# Autodesk Inventor assembly: DD_KVD_002_B
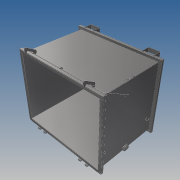
[picture p0: Inventor's stored thumbnail of the model, 180x180]
Saved by Autodesk Inventor 2017.3 (Build 213256000, 256)
## iProperties
Created: 2023-12-07
Part Number: DD_KVD_002_B
Document SubType Name: Weldment
Designer: Darena
Weld Material: Nerezová ocel, kartáčovaná
Author: Darena
## Documents named in this file (18)
- D:\2_Darena\1_Soukrome\02_Inventor soukromé\Dílna RAKO3\Záhora\Pivovar KONTEJNER\S výklopným dnem\DD_KVD_001\DD_KVD_002_B.iam
- D:\2_Darena\1_Soukrome\02_Inventor soukromé\Dílna RAKO3\Záhora\Pivovar KONTEJNER\S výklopným dnem\DD_KVD_001\DD_KVD_002_01.ipt
- D:\2_Darena\1_Soukrome\02_Inventor soukromé\Dílna RAKO3\Záhora\Pivovar KONTEJNER\S výklopným dnem\DD_KVD_001\DD_KVD_002_02.ipt
- D:\2_Darena\1_Soukrome\02_Inventor soukromé\Dílna RAKO3\Záhora\Pivovar KONTEJNER\S výklopným dnem\DD_KVD_001\DD_KVD_002_05.ipt
- D:\2_Darena\1_Soukrome\02_Inventor soukromé\Dílna RAKO3\Záhora\Pivovar KONTEJNER\S výklopným dnem\DD_KVD_001\DD_KVD_002_03.ipt
- D:\2_Darena\1_Soukrome\02_Inventor soukromé\Dílna RAKO3\Záhora\Pivovar KONTEJNER\S výklopným dnem\DD_KVD_001\DD_KVD_002_04.ipt
- D:\2_Darena\1_Soukrome\02_Inventor soukromé\Dílna RAKO3\Záhora\Pivovar KONTEJNER\S výklopným dnem\DD_KVD_001\DD_KVD_003_10_A.ipt
- D:\2_Darena\1_Soukrome\02_Inventor soukromé\Dílna RAKO3\Záhora\Pivovar KONTEJNER\S výklopným dnem\DD_KVD_001\DD_KVD_002_06.ipt
- D:\2_Darena\1_Soukrome\02_Inventor soukromé\Dílna RAKO3\Záhora\Pivovar KONTEJNER\S výklopným dnem\DD_KVD_001\DD_KVD_002_07.ipt
- D:\2_Darena\1_Soukrome\02_Inventor soukromé\Dílna RAKO3\Záhora\Pivovar KONTEJNER\S výklopným dnem\DD_KVD_001\DD_KVD_002_08.ipt
- D:\2_Darena\1_Soukrome\02_Inventor soukromé\Dílna RAKO3\Záhora\Pivovar KONTEJNER\S výklopným dnem\DD_KVD_001\DD_KVD_002_09.ipt
- D:\2_Darena\1_Soukrome\02_Inventor soukromé\Dílna RAKO3\Záhora\Pivovar KONTEJNER\S výklopným dnem\DD_KVD_001\DD_KVD_002_10.ipt
- D:\2_Darena\1_Soukrome\02_Inventor soukromé\Dílna RAKO3\Záhora\Pivovar KONTEJNER\S výklopným dnem\DD_KVD_001\DD_KVD_002_11.ipt
- D:\2_Darena\1_Soukrome\02_Inventor soukromé\Dílna RAKO3\Záhora\Pivovar KONTEJNER\S výklopným dnem\DD_KVD_001\ZA_VK_010.iam
- D:\2_Darena\1_Soukrome\02_Inventor soukromé\Dílna RAKO3\Záhora\Pivovar KONTEJNER\S výklopným dnem\DD_KVD_001\DD_KVD_002_13.ipt
- D:\2_Darena\1_Soukrome\02_Inventor soukromé\Dílna RAKO3\Záhora\Pivovar KONTEJNER\S výklopným dnem\DD_KVD_001\DD_KVD_002_12.ipt
- D:\2_Darena\1_Soukrome\02_Inventor soukromé\Dílna RAKO3\Záhora\Pivovar KONTEJNER\S výklopným dnem\DD_KVD_001\DD_KVD_002_14.ipt
- D:\2_Darena\1_Soukrome\02_Inventor soukromé\Dílna RAKO3\Záhora\Pivovar KONTEJNER\S výklopným dnem\DD_KVD_001\DD_KVD_004.iam
## Components (38 placed, 17 different names)
1. DD_KVD_002_01:1 — Stejný směr:7, Proti sobě:65, Proti sobě:69, Proti sobě:71, Proti sobě:72, Stejný směr:11, Stejný směr:12, Proti sobě:84, Proti sobě:86, Stejný směr:21, Proti sobě:101, Proti sobě:103, Proti sobě:105, Stejný směr:29, Proti sobě:128, Úhel:7
2. DD_KVD_002_01:2 — Proti sobě:63, Proti sobě:66, Proti sobě:67, Proti sobě:74, Stejný směr:13, Proti sobě:121, Proti sobě:124, Stejný směr:32, Stejný směr:39
3. DD_KVD_002_02:2 — Stejný směr:6, Proti sobě:65, Proti sobě:66, Stejný směr:12, Stejný směr:13, Proti sobě:90, Proti sobě:118, Proti sobě:122, Stejný směr:31, Proti sobě:130, Proti sobě:132, Proti sobě:133
4. DD_KVD_002_02:3 — Proti sobě:64, Proti sobě:67, Proti sobě:70, Stejný směr:11, Úhel:3, Úhel:4, Proti sobě:127, Proti sobě:131
5. DD_KVD_002_03:1 — Stejný směr:3, Proti sobě:57, Proti sobě:58, Stejný směr:4, Proti sobě:59
6. DD_KVD_002_03:2 — Stejný směr:5, Proti sobě:61, Proti sobě:62, Proti sobě:70
7. DD_KVD_002_03:3 — Stejný směr:17, Proti sobě:90, Proti sobě:97, Stejný směr:23, Proti sobě:129, Proti sobě:134
8. DD_KVD_002_03:4 — Proti sobě:85, Stejný směr:16, Proti sobě:99, Stejný směr:24, Stejný směr:33, Stejný směr:36
9. DD_KVD_002_04:1 — Stejný směr:4, Proti sobě:59, Stejný směr:5, Proti sobě:75, Proti sobě:123, Proti sobě:126
10. DD_KVD_002_04:2 — Stejný směr:3, Proti sobě:57, Proti sobě:58, Proti sobě:61, Proti sobě:62, Proti sobě:69, Proti sobě:71, Proti sobě:73
11. DD_KVD_002_04:3 — Proti sobě:91, Proti sobě:92, Proti sobě:93, Proti sobě:94, Proti sobě:95, Stejný směr:37
12. DD_KVD_002_04:4 — Proti sobě:84, Proti sobě:85, Stejný směr:16, Stejný směr:17, Proti sobě:86, Proti sobě:100, Proti sobě:102, Proti sobě:104, HÁK ZAJIŠTĚNÝ, Proti sobě:119
13. DD_KVD_003_10_A:1 — Proti sobě:91, Stejný směr:20, Proti sobě:95, Proti sobě:96
14. DD_KVD_003_10_A:2 — Proti sobě:92, Stejný směr:19, Stejný směr:20, Proti sobě:96, Proti sobě:97
15. DD_KVD_003_10_A:3 — Proti sobě:93, Stejný směr:18, Proti sobě:98
16. DD_KVD_003_10_A:4 — Proti sobě:94, Stejný směr:18, Stejný směr:19, Proti sobě:98, Proti sobě:99
17. DD_KVD_002_06:1 — Proti sobě:100, Proti sobě:101, Stejný směr:23, Proti sobě:106, Proti sobě:107
18. DD_KVD_002_06:2 — Stejný směr:22, Proti sobě:102, Proti sobě:103, Proti sobě:110
19. DD_KVD_002_06:3 — Proti sobě:104, Proti sobě:105, Stejný směr:24, Proti sobě:108, Proti sobě:109
20. DD_KVD_002_07:1 — Proti sobě:106, Proti sobě:107, Stejný směr:25, Úhel:1, HÁK ZAJIŠTĚNÝ, Úhel:5
21. DD_KVD_002_07:2 — Proti sobě:108, Proti sobě:109, Stejný směr:25, Úhel:2
22. DD_KVD_002_08:1 — Proti sobě:110, Stejný směr:26, Úhel:1, Proti sobě:112, Stejný směr:27, Proti sobě:113, Stejný směr:28
23. DD_KVD_002_09:1 — Proti sobě:112, Stejný směr:27, Úhel:5, Úhel:6
24. DD_KVD_002_10:1 — Proti sobě:113, Stejný směr:28, Úhel:2
25. ZA_VK_010:1 [sub-assembly] — Úhel:3, Úhel:4, Tečnost:4, Stejný směr:34
26. DD_KVD_002_13:1 — Proti sobě:118, Proti sobě:119, Stejný směr:29, Proti sobě:120, Tečnost:3
27. DD_KVD_002_12:1 — Proti sobě:120, Tečnost:3, Úhel:6, Proti sobě:132, Úhel:7
28. DD_KVD_002_14:1 — Proti sobě:124, Proti sobě:125, Proti sobě:126, Stejný směr:30
29. DD_KVD_002_14:2 — Stejný směr:30, Stejný směr:31, Stejný směr:32
30. DD_KVD_002_14:3 — Proti sobě:121, Proti sobě:122, Proti sobě:123, Proti sobě:125
31. DD_KVD_002_11:1 — Proti sobě:127, Proti sobě:128, Stejný směr:33, Tečnost:4, Stejný směr:34
32. DD_KVD_002_14:4 — Stejný směr:36, Proti sobě:131, Stejný směr:37, Stejný směr:38
33. DD_KVD_002_14:5 — Proti sobě:129, Proti sobě:130, Stejný směr:38
34. DD_KVD_004:1 [sub-assembly] — Proti sobě:133, Stejný směr:39, Proti sobě:134
35. DD_KVD_002_05:5 — Proti sobě:72, Proti sobě:73, Stejný směr:9, Stejný směr:10
36. DD_KVD_002_05:6 — Proti sobě:74, Proti sobě:75, Stejný směr:9
37. DD_KVD_002_05:7
38. DD_KVD_002_05:8
## Component patterns: (2 elements, first: DD_KVD_002_05:5 + DD_KVD_002_05:6)
## Relationships (108: Mate 64, Flush 35, Angle 7, Tangent 2)
- Proti sobě:63 [Mate]: DD_KVD_002_01:2
- Stejný směr:3 [Flush]: DD_KVD_002_03:1 ↔ DD_KVD_002_04:2
- Proti sobě:57 [Mate]: DD_KVD_002_03:1 ↔ DD_KVD_002_04:2
- Proti sobě:58 [Mate]: DD_KVD_002_03:1 ↔ DD_KVD_002_04:2
- Stejný směr:4 [Flush]: DD_KVD_002_03:1 ↔ DD_KVD_002_04:1
- Proti sobě:59 [Mate]: DD_KVD_002_03:1 ↔ DD_KVD_002_04:1
- Stejný směr:5 [Flush]: DD_KVD_002_03:2 ↔ DD_KVD_002_04:1
- Proti sobě:61 [Mate]: DD_KVD_002_03:2 ↔ DD_KVD_002_04:2
- Proti sobě:62 [Mate]: DD_KVD_002_03:2 ↔ DD_KVD_002_04:2
- Proti sobě:64 [Mate]: DD_KVD_002_02:3
- Stejný směr:6 [Flush]: DD_KVD_002_02:2
- Stejný směr:7 [Flush]: DD_KVD_002_01:1
- Proti sobě:65 [Mate]: DD_KVD_002_01:1 ↔ DD_KVD_002_02:2
- Proti sobě:66 [Mate]: DD_KVD_002_01:2 ↔ DD_KVD_002_02:2
- Proti sobě:67 [Mate]: DD_KVD_002_01:2 ↔ DD_KVD_002_02:3
- Proti sobě:69 [Mate]: DD_KVD_002_01:1 ↔ DD_KVD_002_04:2
- Proti sobě:70 [Mate]: DD_KVD_002_02:3 ↔ DD_KVD_002_03:2
- Proti sobě:71 [Mate]: DD_KVD_002_01:1 ↔ DD_KVD_002_04:2
- Proti sobě:72 [Mate]: DD_KVD_002_01:1 ↔ DD_KVD_002_05:5
- Proti sobě:73 [Mate]: DD_KVD_002_04:2 ↔ DD_KVD_002_05:5
- Proti sobě:74 [Mate]: DD_KVD_002_01:2 ↔ DD_KVD_002_05:6
- Proti sobě:75 [Mate]: DD_KVD_002_04:1 ↔ DD_KVD_002_05:6
- Stejný směr:9 [Flush]: DD_KVD_002_05:5 ↔ DD_KVD_002_05:6
- Stejný směr:10 [Flush] (380 mm): DD_KVD_002_05:5
- Stejný směr:11 [Flush]: DD_KVD_002_01:1 ↔ DD_KVD_002_02:3
- Stejný směr:12 [Flush]: DD_KVD_002_01:1 ↔ DD_KVD_002_02:2
- Stejný směr:13 [Flush]: DD_KVD_002_01:2 ↔ DD_KVD_002_02:2
- [Flush]: DD_KVD_002_03:3 ↔ DD_KVD_002_04:4
- [Mate]: DD_KVD_002_03:3 ↔ DD_KVD_002_04:4
- [Mate]: DD_KVD_002_03:3 ↔ DD_KVD_002_04:4
- [Flush]: DD_KVD_002_03:3 ↔ DD_KVD_002_04:3
- [Mate]: DD_KVD_002_03:3 ↔ DD_KVD_002_04:3
- Proti sobě:84 [Mate]: DD_KVD_002_01:1 ↔ DD_KVD_002_04:4
- Proti sobě:85 [Mate]: DD_KVD_002_03:4 ↔ DD_KVD_002_04:4
- Stejný směr:16 [Flush]: DD_KVD_002_03:4 ↔ DD_KVD_002_04:4
- Stejný směr:17 [Flush]: DD_KVD_002_03:3 ↔ DD_KVD_002_04:4
- Proti sobě:86 [Mate]: DD_KVD_002_01:1 ↔ DD_KVD_002_04:4
- Proti sobě:90 [Mate]: DD_KVD_002_02:2 ↔ DD_KVD_002_03:3
- Proti sobě:91 [Mate]: DD_KVD_002_04:3 ↔ DD_KVD_003_10_A:1
- Proti sobě:92 [Mate]: DD_KVD_002_04:3 ↔ DD_KVD_003_10_A:2
- Proti sobě:93 [Mate]: DD_KVD_002_04:3 ↔ DD_KVD_003_10_A:3
- Proti sobě:94 [Mate]: DD_KVD_002_04:3 ↔ DD_KVD_003_10_A:4
- Stejný směr:18 [Flush]: DD_KVD_003_10_A:3 ↔ DD_KVD_003_10_A:4
- Stejný směr:19 [Flush]: DD_KVD_003_10_A:2 ↔ DD_KVD_003_10_A:4
- Stejný směr:20 [Flush]: DD_KVD_003_10_A:1 ↔ DD_KVD_003_10_A:2
- Proti sobě:95 [Mate]: DD_KVD_002_04:3 ↔ DD_KVD_003_10_A:1
- Proti sobě:96 [Mate] (61 mm): DD_KVD_003_10_A:1 ↔ DD_KVD_003_10_A:2
- Proti sobě:97 [Mate] (-285 mm): DD_KVD_002_03:3 ↔ DD_KVD_003_10_A:2
- Proti sobě:98 [Mate] (61 mm): DD_KVD_003_10_A:3 ↔ DD_KVD_003_10_A:4
- Proti sobě:99 [Mate] (-285 mm): DD_KVD_002_03:4 ↔ DD_KVD_003_10_A:4
- Stejný směr:21 [Flush]: DD_KVD_002_01:1
- Proti sobě:100 [Mate]: DD_KVD_002_04:4 ↔ DD_KVD_002_06:1
- Proti sobě:101 [Mate]: DD_KVD_002_01:1 ↔ DD_KVD_002_06:1
- Stejný směr:22 [Flush] (-3 mm): DD_KVD_002_06:2
- Proti sobě:102 [Mate]: DD_KVD_002_04:4 ↔ DD_KVD_002_06:2
- Proti sobě:103 [Mate]: DD_KVD_002_01:1 ↔ DD_KVD_002_06:2
- Proti sobě:104 [Mate]: DD_KVD_002_04:4 ↔ DD_KVD_002_06:3
- Proti sobě:105 [Mate]: DD_KVD_002_01:1 ↔ DD_KVD_002_06:3
- Stejný směr:23 [Flush] (150 mm): DD_KVD_002_03:3 ↔ DD_KVD_002_06:1
- Stejný směr:24 [Flush] (-150 mm): DD_KVD_002_03:4 ↔ DD_KVD_002_06:3
- Proti sobě:106 [Mate] (3 mm): DD_KVD_002_06:1 ↔ DD_KVD_002_07:1
- Proti sobě:107 [Mate]: DD_KVD_002_06:1 ↔ DD_KVD_002_07:1
- Proti sobě:108 [Mate] (3 mm): DD_KVD_002_06:3 ↔ DD_KVD_002_07:2
- Proti sobě:109 [Mate]: DD_KVD_002_06:3 ↔ DD_KVD_002_07:2
- Stejný směr:25 [Flush]: DD_KVD_002_07:1 ↔ DD_KVD_002_07:2
- Proti sobě:110 [Mate]: DD_KVD_002_06:2 ↔ DD_KVD_002_08:1
- Stejný směr:26 [Flush]: DD_KVD_002_08:1
- Úhel:1 [Angle] (0 deg): DD_KVD_002_07:1 ↔ DD_KVD_002_08:1
- HÁK ZAJIŠTĚNÝ [Mate]: DD_KVD_002_04:4 ↔ DD_KVD_002_07:1
- Proti sobě:112 [Mate]: DD_KVD_002_08:1 ↔ DD_KVD_002_09:1
- Stejný směr:27 [Flush] (5 mm): DD_KVD_002_08:1 ↔ DD_KVD_002_09:1
- Proti sobě:113 [Mate]: DD_KVD_002_08:1 ↔ DD_KVD_002_10:1
- Stejný směr:28 [Flush] (-5 mm): DD_KVD_002_08:1 ↔ DD_KVD_002_10:1
- Úhel:2 [Angle] (0 deg): DD_KVD_002_07:2 ↔ DD_KVD_002_10:1
- Úhel:3 [Angle] (0 deg): DD_KVD_002_02:3 ↔ ZA_VK_010:1
- Úhel:4 [Angle] (0 deg): DD_KVD_002_02:3 ↔ ZA_VK_010:1
- Úhel:5 [Angle] (0 deg): DD_KVD_002_07:1 ↔ DD_KVD_002_09:1
- Proti sobě:118 [Mate]: DD_KVD_002_02:2 ↔ DD_KVD_002_13:1
- Proti sobě:119 [Mate] (345 mm): DD_KVD_002_04:4 ↔ DD_KVD_002_13:1
- Stejný směr:29 [Flush] (19.5 mm): DD_KVD_002_01:1 ↔ DD_KVD_002_13:1
- Proti sobě:120 [Mate]: DD_KVD_002_13:1 ↔ DD_KVD_002_12:1
- Tečnost:3 [Tangent]: DD_KVD_002_13:1 ↔ DD_KVD_002_12:1
- Úhel:6 [Angle] (180 deg): DD_KVD_002_09:1 ↔ DD_KVD_002_12:1
- Proti sobě:121 [Mate]: DD_KVD_002_01:2 ↔ DD_KVD_002_14:3
- Proti sobě:122 [Mate] (-187 mm): DD_KVD_002_02:2 ↔ DD_KVD_002_14:3
- Proti sobě:123 [Mate] (75 mm): DD_KVD_002_04:1 ↔ DD_KVD_002_14:3
- Proti sobě:124 [Mate] (17.5 mm): DD_KVD_002_01:2 ↔ DD_KVD_002_14:1
- Proti sobě:125 [Mate] (-129 mm): DD_KVD_002_14:1 ↔ DD_KVD_002_14:3
- Proti sobě:126 [Mate] (55 mm): DD_KVD_002_04:1 ↔ DD_KVD_002_14:1
- Stejný směr:30 [Flush]: DD_KVD_002_14:1 ↔ DD_KVD_002_14:2
- Stejný směr:31 [Flush] (17.5 mm): DD_KVD_002_02:2 ↔ DD_KVD_002_14:2
- Stejný směr:32 [Flush] (200 mm): DD_KVD_002_01:2 ↔ DD_KVD_002_14:2
- Proti sobě:127 [Mate]: DD_KVD_002_02:3 ↔ DD_KVD_002_11:1
- Proti sobě:128 [Mate] (-105 mm): DD_KVD_002_01:1 ↔ DD_KVD_002_11:1
- Stejný směr:33 [Flush] (308 mm): DD_KVD_002_03:4 ↔ DD_KVD_002_11:1
- Tečnost:4 [Tangent]: ZA_VK_010:1 ↔ DD_KVD_002_11:1
- Stejný směr:34 [Flush]: ZA_VK_010:1 ↔ DD_KVD_002_11:1
- Proti sobě:129 [Mate] (3 mm): DD_KVD_002_03:3 ↔ DD_KVD_002_14:5
- Proti sobě:130 [Mate] (6 mm): DD_KVD_002_02:2 ↔ DD_KVD_002_14:5
- Stejný směr:36 [Flush] (-3 mm): DD_KVD_002_03:4 ↔ DD_KVD_002_14:4
- Proti sobě:131 [Mate] (6 mm): DD_KVD_002_02:3 ↔ DD_KVD_002_14:4
- Stejný směr:37 [Flush] (-260 mm): DD_KVD_002_04:3 ↔ DD_KVD_002_14:4
- Stejný směr:38 [Flush]: DD_KVD_002_14:4 ↔ DD_KVD_002_14:5
- Proti sobě:132 [Mate] (6 mm): DD_KVD_002_02:2 ↔ DD_KVD_002_12:1
- Úhel:7 [Angle] (0 deg): DD_KVD_002_01:1 ↔ DD_KVD_002_12:1
- Proti sobě:133 [Mate]: DD_KVD_002_02:2 ↔ DD_KVD_004:1
- Stejný směr:39 [Flush] (10 mm): DD_KVD_002_01:2 ↔ DD_KVD_004:1
- Proti sobě:134 [Mate] (300 mm): DD_KVD_002_03:3 ↔ DD_KVD_004:1
## Named parameters: d210_d176 = 0 mm, d211_d177 = 0 mm, d215_d173 = 0 mm, d216_d174 = 0 mm, d217_d175 = 0 mm
